# Autodesk Inventor assembly: Ensamble total
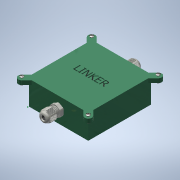
[picture p0: Inventor's stored thumbnail of the model, 180x180]
Saved by Autodesk Inventor 2021 (Build 250183000, 183)
## iProperties
Created: 2021-03-04
Part Number: Ensamble total
Material: Generic
Document SubType Name: Assembly
Designer: Usuario
Author: Usuario
## Documents named in this file (7)
- C:\Users\Usuario\Desktop\INVENTOR\Ensamble total.iam
- C:\Users\Usuario\Desktop\INVENTOR\Base inferior.ipt
- C:\Users\Usuario\Desktop\INVENTOR\Ensamble base + comp.iam
- C:\Users\Usuario\Desktop\INVENTOR\PG7 Cable Gland.ipt
- C:\Users\Usuario\Desktop\INVENTOR\tapa.ipt
- C:\Users\Usuario\Documents\Inventor\Content Center Files\R2021\en-US\AS 1427(06)\AS 1427 - M3 x 10(5) III.ipt
- C:\Users\Usuario\Documents\Inventor\Content Center Files\R2021\en-US\AS 1474(1)\AS 1474 - M3(1).ipt
## Components (13 placed, 6 different names)
1. Base inferior:1 — Insert:1, Insert:3, Insert:4, Insert:5, Insert:10, Insert:11, Insert:12, Insert:13
2. Ensamble base + comp:1 [sub-assembly] — Insert:1
3. PG7 Cable Gland:1 — Insert:4
4. PG7 Cable Gland:2 — Insert:3
5. tapa:1 — Insert:5, Insert:6, Insert:7, Insert:8, Insert:9
6. AS 1427 H Raised - Metric M3 x 10:1 — Insert:7
7. AS 1427 H Raised - Metric M3 x 10:2 — Insert:8
8. AS 1427 H Raised - Metric M3 x 10:3 — Insert:6
9. AS 1427 H Raised - Metric M3 x 10:4 — Insert:9
10. AS 1474 - Metric M3:1 — Insert:12
11. AS 1474 - Metric M3:2 — Insert:13
12. AS 1474 - Metric M3:3 — Insert:11
13. AS 1474 - Metric M3:4 — Insert:10
## Relationships (12: Insert 12)
- Insert:1: Base inferior:1 ↔ Ensamble base + comp:1
- Insert:3: Base inferior:1 ↔ PG7 Cable Gland:2
- Insert:4: Base inferior:1 ↔ PG7 Cable Gland:1
- Insert:5: Base inferior:1 ↔ tapa:1
- Insert:6: tapa:1 ↔ AS 1427 H Raised - Metric M3 x 10:3
- Insert:7: tapa:1 ↔ AS 1427 H Raised - Metric M3 x 10:1
- Insert:8: tapa:1 ↔ AS 1427 H Raised - Metric M3 x 10:2
- Insert:9: tapa:1 ↔ AS 1427 H Raised - Metric M3 x 10:4
- Insert:10: Base inferior:1 ↔ AS 1474 - Metric M3:4
- Insert:11: Base inferior:1 ↔ AS 1474 - Metric M3:3
- Insert:12: Base inferior:1 ↔ AS 1474 - Metric M3:1
- Insert:13: Base inferior:1 ↔ AS 1474 - Metric M3:2
